# Autodesk Inventor assembly: EndEffectorAssembly
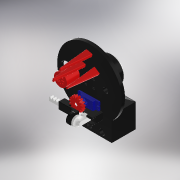
[picture p0: Inventor's stored thumbnail of the model, 180x180]
Saved by Autodesk Inventor 2020.3 (Build 243373000, 373)
## iProperties
Created: 2021-08-11
Part Number: EndEffectorAssembly
Document SubType Name: Assembly
Designer: justi
Mass: 134.462 g
Surface Area: 641.511 cm^2
Volume: 125.455 cm^3
Density: 1.07179 g/cm^3
Author: justi
## Documents named in this file (9)
- F:\UQ Engineering\2021 ~ 5th Year\Semester 2\METR4911-THESIS\FarmBot CAD\FarmBotV1\EndEffectorAssembly.iam
- F:\UQ Engineering\2021 ~ 5th Year\Semester 2\METR4911-THESIS\FarmBot CAD\FarmBotV1\EndEffectorPlate.ipt
- F:\UQ Engineering\2021 ~ 5th Year\Semester 2\METR4911-THESIS\FarmBot CAD\FarmBotV1\tower-pro-sg90-micro-servo\microservoAssembly.iam
- F:\UQ Engineering\2021 ~ 5th Year\Semester 2\METR4911-THESIS\FarmBot CAD\FarmBotV1\EndEffectorJoint.ipt
- F:\UQ Engineering\2021 ~ 5th Year\Semester 2\METR4911-THESIS\FarmBot CAD\FarmBotV1\EndEffectorRotational.ipt
- F:\UQ Engineering\2021 ~ 5th Year\Semester 2\METR4911-THESIS\FarmBot CAD\FarmBotV1\EndEffectorAssembly\Design Accelerator\Spur Gears2.iam
- F:\UQ Engineering\2021 ~ 5th Year\Semester 2\METR4911-THESIS\FarmBot CAD\FarmBotV1\tower-pro-sg90-micro-servo\Rackv1.ipt
- F:\UQ Engineering\2021 ~ 5th Year\Semester 2\METR4911-THESIS\FarmBot CAD\FarmBotV1\tower-pro-sg90-micro-servo\WeedingTeeth.ipt
- F:\UQ Engineering\2021 ~ 5th Year\Semester 2\METR4911-THESIS\FarmBot CAD\FarmBotV1\tower-pro-sg90-micro-servo\DiffusionModule.ipt
## Components (10 placed, 8 different names)
1. EndEffectorJoint:1
2. EndEffectorRotational:1
3. EndEffectorPlate:1 — Mate:11, Mate:12, Mate:13, Mate:14, Mate:15, Mate:16, Mate:17, Mate:18
4. microservoAssembly:1 [sub-assembly] — Mate:9, Flush:11, Mate:10, Flush:13
5. Spur Gears:1 [sub-assembly] — Mate:9, Flush:11, Mate:10, Flush:12
6. Rackv1:1 — Flush:12, Flush:13
7. WeedingTeeth:1 — Mate:11, Mate:14
8. WeedingTeeth:2 — Mate:12, Mate:16
9. WeedingTeeth:3 — Mate:13, Mate:15
10. DiffusionModule:1 — Mate:17, Mate:18
## Relationships (21: Mate 18, Flush 3)
- [Mate]: EndEffectorJoint:1 ↔ EndEffectorRotational:1
- [Mate]: EndEffectorJoint:1 ↔ EndEffectorRotational:1
- [Mate]: EndEffectorRotational:1 ↔ EndEffectorPlate:1
- [Mate]: EndEffectorRotational:1 ↔ EndEffectorPlate:1
- [Mate]: EndEffectorRotational:1 ↔ EndEffectorPlate:1
- [Mate]: EndEffectorPlate:1 ↔ microservoAssembly:1
- [Mate]: EndEffectorPlate:1 ↔ microservoAssembly:1
- [Mate]: EndEffectorPlate:1 ↔ microservoAssembly:1
- Mate:9: microservoAssembly:1 ↔ Spur Gears:1
- Flush:11: microservoAssembly:1 ↔ Spur Gears:1
- Mate:10: microservoAssembly:1 ↔ Spur Gears:1
- Flush:12: Spur Gears:1 ↔ Rackv1:1
- Flush:13 (-8.5 mm): microservoAssembly:1 ↔ Rackv1:1
- Mate:11: EndEffectorPlate:1 ↔ WeedingTeeth:1
- Mate:12: EndEffectorPlate:1 ↔ WeedingTeeth:2
- Mate:13: EndEffectorPlate:1 ↔ WeedingTeeth:3
- Mate:14: EndEffectorPlate:1 ↔ WeedingTeeth:1
- Mate:15: EndEffectorPlate:1 ↔ WeedingTeeth:3
- Mate:16: EndEffectorPlate:1 ↔ WeedingTeeth:2
- Mate:17: EndEffectorPlate:1 ↔ DiffusionModule:1
- Mate:18: EndEffectorPlate:1 ↔ DiffusionModule:1
